# Autodesk Inventor assembly: new metal drivetrain motor mount_MIR
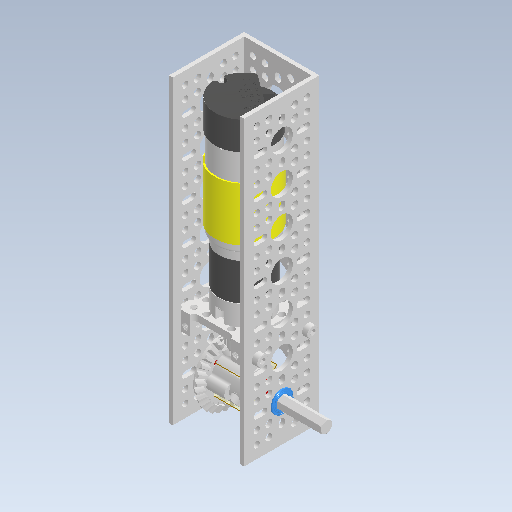
[picture p0: Inventor's stored thumbnail of the model, 512x512]
Saved by Autodesk Inventor 2020 (Build 240168000, 168)
## iProperties
Created: 2020-02-22
Part Number: new metal drivetrain motor mount_MIR
Document SubType Name: Assembly
Designer: jackm
Author: jackm
## Documents named in this file (10)
- D:\FTC8863\2019 Robot\Mecanum Drive Train Metal\new metal drivetrain motor mount_MIR.iam
- D:\FTC8863\GoBilda\1309 Parts\2102-0008-0090_MIR.ipt
- D:\FTC8863\GoBilda\3204 Parts\1120-0007-0192_MIR.ipt
- D:\FTC8863\GoBilda\1201 Parts\1201-0043-0002_MIR.ipt
- D:\FTC8863\GoBilda\5202 Parts\5202-0002-0014 part_MIR.ipt
- D:\FTC8863\StepLibraries\Screws\M4 x 10 SOCKET HEAD CAP SCREW_MIR.ipt
- D:\FTC8863\StepLibraries\Screws\M4 x 12 SOCKET HEAD CAP SCREW_MIR.ipt
- D:\FTC8863\2019 Robot\Generic Parts\Gobilda bevel gears + 8mm REX hyper hub_MIR.iam
- D:\FTC8863\GoBilda\1601 Parts\1601-0014-0008_MIR.ipt
- D:\FTC8863\2019 Robot\Mecanum Drive Train Metal\spacer for channel inside_MIR.ipt
## Components (14 placed, 9 different names)
1. 2102-0008-0090_MIR:1 — Mate:47, Mate:51, Mate:49, Mate:55, Mate:57
2. 1120-0007-0192_MIR:1 — Mate:35, Mate:34, Mate:33, Mate:37, Mate:41, Mate:40, Mate:43, Mate:42, Mate:38, Mate:36, Mate:58, Mate:50, Mate:59, Mate:48
3. 1201-0043-0002_MIR:1 — Mate:35, Mate:34, Mate:33, Mate:32, Mate:31, Mate:30, Mate:29, Mate:39, Mate:44
4. 5202-0002-0014 part_MIR:1 — Mate:32, Mate:31, Mate:30, Mate:29, Mate:45, Mate:46
5. M4 x 10 SOCKET HEAD CAP SCREW_MIR:1 — Mate:39, Mate:37
6. M4 x 10 SOCKET HEAD CAP SCREW_MIR:2 — Mate:41, Mate:40
7. M4 x 10 SOCKET HEAD CAP SCREW_MIR:3 — Mate:43, Mate:42
8. M4 x 10 SOCKET HEAD CAP SCREW_MIR:4 — Mate:38, Mate:36
9. M4 x 12 SOCKET HEAD CAP SCREW_MIR:1 — Mate:45, Mate:44
10. Gobilda bevel gears + 8mm REX hyper hub_MIR:1 [sub-assembly] — Mate:47, Mate:46, Mate:56
11. 1601-0014-0008_MIR:1 — Mate:58, Mate:51, Mate:50
12. 1601-0014-0008_MIR:2 — Mate:59, Mate:48, Mate:49, Mate:54
13. spacer for channel inside_MIR:1 — Mate:54, Mate:55
14. spacer for channel inside_MIR:2 — Mate:57, Mate:56
## Relationships (29: Mate 29)
- Mate:35: 1120-0007-0192_MIR:1 ↔ 1201-0043-0002_MIR:1
- Mate:34: 1120-0007-0192_MIR:1 ↔ 1201-0043-0002_MIR:1
- Mate:33: 1120-0007-0192_MIR:1 ↔ 1201-0043-0002_MIR:1
- Mate:32: 1201-0043-0002_MIR:1 ↔ 5202-0002-0014 part_MIR:1
- Mate:31: 1201-0043-0002_MIR:1 ↔ 5202-0002-0014 part_MIR:1
- Mate:30: 1201-0043-0002_MIR:1 ↔ 5202-0002-0014 part_MIR:1
- Mate:29: 1201-0043-0002_MIR:1 ↔ 5202-0002-0014 part_MIR:1
- Mate:39: 1201-0043-0002_MIR:1 ↔ M4 x 10 SOCKET HEAD CAP SCREW_MIR:1
- Mate:37: 1120-0007-0192_MIR:1 ↔ M4 x 10 SOCKET HEAD CAP SCREW_MIR:1
- Mate:41: 1120-0007-0192_MIR:1 ↔ M4 x 10 SOCKET HEAD CAP SCREW_MIR:2
- Mate:40: 1120-0007-0192_MIR:1 ↔ M4 x 10 SOCKET HEAD CAP SCREW_MIR:2
- Mate:43: 1120-0007-0192_MIR:1 ↔ M4 x 10 SOCKET HEAD CAP SCREW_MIR:3
- Mate:42: 1120-0007-0192_MIR:1 ↔ M4 x 10 SOCKET HEAD CAP SCREW_MIR:3
- Mate:38: 1120-0007-0192_MIR:1 ↔ M4 x 10 SOCKET HEAD CAP SCREW_MIR:4
- Mate:36: 1120-0007-0192_MIR:1 ↔ M4 x 10 SOCKET HEAD CAP SCREW_MIR:4
- Mate:45: 5202-0002-0014 part_MIR:1 ↔ M4 x 12 SOCKET HEAD CAP SCREW_MIR:1
- Mate:44: 1201-0043-0002_MIR:1 ↔ M4 x 12 SOCKET HEAD CAP SCREW_MIR:1
- Mate:47: 2102-0008-0090_MIR:1 ↔ Gobilda bevel gears + 8mm REX hyper hub_MIR:1
- Mate:46: 5202-0002-0014 part_MIR:1 ↔ Gobilda bevel gears + 8mm REX hyper hub_MIR:1
- Mate:58: 1120-0007-0192_MIR:1 ↔ 1601-0014-0008_MIR:1
- Mate:51: 2102-0008-0090_MIR:1 ↔ 1601-0014-0008_MIR:1
- Mate:50: 1120-0007-0192_MIR:1 ↔ 1601-0014-0008_MIR:1
- Mate:59: 1120-0007-0192_MIR:1 ↔ 1601-0014-0008_MIR:2
- Mate:48: 1120-0007-0192_MIR:1 ↔ 1601-0014-0008_MIR:2
- Mate:49: 2102-0008-0090_MIR:1 ↔ 1601-0014-0008_MIR:2
- Mate:54: 1601-0014-0008_MIR:2 ↔ spacer for channel inside_MIR:1
- Mate:55: 2102-0008-0090_MIR:1 ↔ spacer for channel inside_MIR:1
- Mate:57: 2102-0008-0090_MIR:1 ↔ spacer for channel inside_MIR:2
- Mate:56: Gobilda bevel gears + 8mm REX hyper hub_MIR:1 ↔ spacer for channel inside_MIR:2
